# Autodesk Inventor assembly: PreFoldedBody
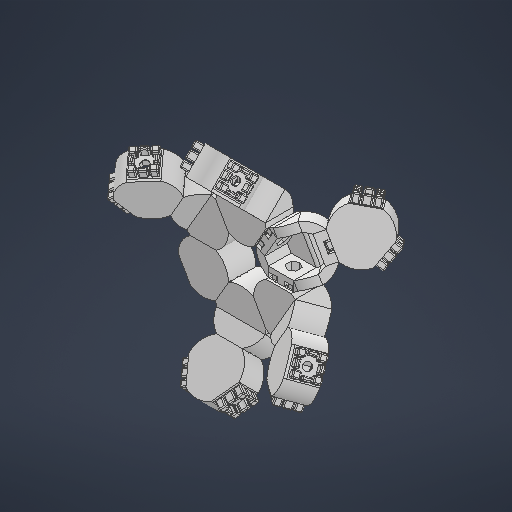
[picture p0: Inventor's stored thumbnail of the model, 512x512]
Saved by Autodesk Inventor 2026.2 (Build 302298000, 298)
## iProperties
Created: 2026-04-30
Part Number: PreFoldedBody
Document SubType Name: Assembly
Designer: Jakub Schmidt
Author: Jakub Schmidt
## Documents named in this file (7)
- C:\Users\Jakub Schmidt\Desktop\100M_SA\SG\10mm (Recent)\2x2mm(Recent)\2DFolded\BeetleDarhani\BeetleFold.iam
- C:\Users\Jakub Schmidt\Desktop\100M_SA\SG\10mm (Recent)\2x2mm(Recent)\2DFolded\BeetleDarhani\BodyFoldedSide1.ipt
- C:\Users\Jakub Schmidt\Desktop\100M_SA\SG\10mm (Recent)\2x2mm(Recent)\2DFolded\BeetleDarhani\BodyFoldedSide2.ipt
- C:\Users\Jakub Schmidt\Desktop\100M_SA\SG\10mm (Recent)\2x2mm(Recent)\2DFolded\BeetleDarhani\SGA.ipt
- C:\Users\Jakub Schmidt\Desktop\100M_SA\SG\10mm (Recent)\2x2mm(Recent)\2DFolded\BeetleDarhani\SGB.ipt
- C:\Users\Jakub Schmidt\Desktop\100M_SA\SG\10mm (Recent)\2x2mm(Recent)\2DFolded\BeetleDarhani\Body.ipt
- C:\Users\Jakub Schmidt\Desktop\100M_SA\SG\10mm (Recent)\2x2mm(Recent)\2DFolded\BeetleDarhani\SGX.ipt
## Components (49 placed, 6 different names)
1. BodyFoldedSide1:1 — Mate:1, Mate:2, Mate:3, Mate:16, Mate:17, Mate:18, Flush:1, Mate:78, Mate:79, Mate:80
2. BodyFoldedSide2:1 — Mate:1, Mate:2, Mate:3, Mate:19, Mate:20, Mate:21, Flush:15
3. BodyFoldedSide1:2 — Mate:62, Mate:63, Mate:64, Mate:65, Mate:66, Mate:67
4. BodyFoldedSide2:2 — Mate:85, Mate:86, Mate:87, Flush:10, Flush:11
5. BodyFoldedSide1:3 — Mate:52, Mate:53, Mate:54, Mate:56, Mate:57, Mate:58, Mate:68
6. BodyFoldedSide2:3 — Mate:59, Mate:60, Mate:61, Flush:12
7. BodyFoldedSide1:4 — Mate:22, Mate:23, Mate:24, Flush:1, Mate:26, Mate:27, Mate:30, Flush:3
8. BodyFoldedSide2:4 — Mate:28, Mate:29, Mate:31, Flush:21
9. BodyFoldedSide1:5 — Mate:69, Mate:70, Mate:71, Mate:73, Mate:74, Mate:75
10. BodyFoldedSide2:5 — Mate:82, Mate:83, Mate:84, Flush:19
11. SGA:1 — Flush:2, Mate:78, Mate:79, Mate:80, Mate:81
12. SGB:1 — Mate:16, Mate:17, Mate:18, Mate:77, Flush:9
13. SGB:2 — Mate:19, Mate:20, Mate:21, Flush:14, Mate:117
14. SGB:3 — Mate:22, Mate:23, Mate:24, Flush:2, Mate:81
15. SGA:2 — Mate:26, Mate:27, Mate:30, Mate:41, Flush:4
16. SGA:3 — Mate:28, Mate:29, Mate:31, Flush:20, Mate:138
17. Body:1 — Mate:32, Mate:33, Mate:34, Mate:35, Mate:36, Mate:37, Mate:38, Mate:39, Mate:40, Flush:3
18. SGB:4 — Mate:33, Mate:34, Mate:39, Mate:72, Flush:5, Flush:6
19. SGB:5 — Mate:32, Mate:35, Mate:40, Mate:41, Flush:4
20. SGA:4 — Mate:36, Mate:37, Mate:38
21. SGA:7 — Mate:52, Mate:53, Mate:54, Flush:7, Flush:8, Mate:76
22. SGB:7 — Mate:56, Mate:57, Mate:58
23. SGB:8 — Mate:59, Mate:60, Mate:61, Mate:116, Flush:13
24. SGA:8 — Mate:65, Mate:66, Mate:67, Mate:68
25. SGA:9 — Mate:62, Mate:63, Mate:64, Mate:77, Flush:9
26. SGA:10 — Mate:69, Mate:70, Mate:71, Mate:72, Flush:5, Flush:6
27. SGB:9 — Mate:73, Mate:74, Mate:75, Flush:7, Flush:8, Mate:76
28. SGA:11 — Mate:82, Mate:83, Mate:84, Flush:18, Mate:137
29. SGB:10 — Mate:85, Mate:86, Mate:87, Mate:97
30. Body:2 — Mate:88, Mate:89, Mate:90, Mate:91, Mate:92, Mate:93, Mate:94, Mate:95, Mate:96, Flush:11
31. SGA:12 — Mate:88, Mate:89, Mate:90, Mate:97, Flush:10
32. SGX:1 — Mate:91, Mate:92, Mate:93
33. SGX:2 — Mate:94, Mate:95, Mate:96
34. Body:3 — Flush:12
35. SGA:13 — Mate:116, Flush:13
36. SGX:3
37. SGX:4
38. Body:4 — Flush:15
39. SGA:14 — Flush:14, Mate:117
40. SGX:5
41. SGX:6
42. Body:5 — Mate:127, Mate:128, Flush:16, Flush:19
43. SGX:7
44. SGX:8
45. SGB:11 — Mate:127, Mate:128, Flush:16, Flush:18, Mate:137
46. Body:6 — Flush:21
47. SGX:9
48. SGX:10
49. SGB:12 — Flush:20, Mate:138
## Relationships (144: Mate 123, Flush 21)
- Mate:1: BodyFoldedSide1:1 ↔ BodyFoldedSide2:1
- Mate:2: BodyFoldedSide1:1 ↔ BodyFoldedSide2:1
- Mate:3: BodyFoldedSide1:1 ↔ BodyFoldedSide2:1
- [Mate]: BodyFoldedSide1:2 ↔ BodyFoldedSide2:2
- [Mate]: BodyFoldedSide1:2 ↔ BodyFoldedSide2:2
- [Mate]: BodyFoldedSide1:2 ↔ BodyFoldedSide2:2
- [Mate]: BodyFoldedSide1:3 ↔ BodyFoldedSide2:3
- [Mate]: BodyFoldedSide1:3 ↔ BodyFoldedSide2:3
- [Mate]: BodyFoldedSide1:3 ↔ BodyFoldedSide2:3
- [Mate]: BodyFoldedSide1:4 ↔ BodyFoldedSide2:4
- [Mate]: BodyFoldedSide1:4 ↔ BodyFoldedSide2:4
- [Mate]: BodyFoldedSide1:4 ↔ BodyFoldedSide2:4
- [Mate]: BodyFoldedSide1:5 ↔ BodyFoldedSide2:5
- [Mate]: BodyFoldedSide1:5 ↔ BodyFoldedSide2:5
- [Mate]: BodyFoldedSide1:5 ↔ BodyFoldedSide2:5
- Mate:16: BodyFoldedSide1:1 ↔ SGB:1
- Mate:17: BodyFoldedSide1:1 ↔ SGB:1
- Mate:18: BodyFoldedSide1:1 ↔ SGB:1
- Mate:19: BodyFoldedSide2:1 ↔ SGB:2
- Mate:20: BodyFoldedSide2:1 ↔ SGB:2
- Mate:21: BodyFoldedSide2:1 ↔ SGB:2
- Mate:22: BodyFoldedSide1:4 ↔ SGB:3
- Mate:23: BodyFoldedSide1:4 ↔ SGB:3
- Mate:24: BodyFoldedSide1:4 ↔ SGB:3
- Flush:1: BodyFoldedSide1:1 ↔ BodyFoldedSide1:4
- Flush:2: SGA:1 ↔ SGB:3
- Mate:26: BodyFoldedSide1:4 ↔ SGA:2
- Mate:27: BodyFoldedSide1:4 ↔ SGA:2
- Mate:28: BodyFoldedSide2:4 ↔ SGA:3
- Mate:29: BodyFoldedSide2:4 ↔ SGA:3
- Mate:30: BodyFoldedSide1:4 ↔ SGA:2
- Mate:31: BodyFoldedSide2:4 ↔ SGA:3
- Mate:32: Body:1 ↔ SGB:5
- Mate:33: Body:1 ↔ SGB:4
- Mate:34: Body:1 ↔ SGB:4
- Mate:35: Body:1 ↔ SGB:5
- Mate:36: Body:1 ↔ SGA:4
- Mate:37: Body:1 ↔ SGA:4
- Mate:38: Body:1 ↔ SGA:4
- Mate:39: Body:1 ↔ SGB:4
- Mate:40: Body:1 ↔ SGB:5
- Mate:41: SGA:2 ↔ SGB:5
- Flush:3: BodyFoldedSide1:4 ↔ Body:1
- Flush:4: SGA:2 ↔ SGB:5
- Mate:52: BodyFoldedSide1:3 ↔ SGA:7
- Mate:53: BodyFoldedSide1:3 ↔ SGA:7
- Mate:54: BodyFoldedSide1:3 ↔ SGA:7
- Mate:56: BodyFoldedSide1:3 ↔ SGB:7
- Mate:57: BodyFoldedSide1:3 ↔ SGB:7
- Mate:58: BodyFoldedSide1:3 ↔ SGB:7
- Mate:59: BodyFoldedSide2:3 ↔ SGB:8
- Mate:60: BodyFoldedSide2:3 ↔ SGB:8
- Mate:61: BodyFoldedSide2:3 ↔ SGB:8
- Mate:62: BodyFoldedSide1:2 ↔ SGA:9
- Mate:63: BodyFoldedSide1:2 ↔ SGA:9
- Mate:64: BodyFoldedSide1:2 ↔ SGA:9
- Mate:65: BodyFoldedSide1:2 ↔ SGA:8
- Mate:66: BodyFoldedSide1:2 ↔ SGA:8
- Mate:67: BodyFoldedSide1:2 ↔ SGA:8
- Mate:68: BodyFoldedSide1:3 ↔ SGA:8
- Mate:69: BodyFoldedSide1:5 ↔ SGA:10
- Mate:70: BodyFoldedSide1:5 ↔ SGA:10
- Mate:71: BodyFoldedSide1:5 ↔ SGA:10
- Mate:72: SGB:4 ↔ SGA:10
- Flush:5: SGB:4 ↔ SGA:10
- Flush:6: SGB:4 ↔ SGA:10
- Mate:73: BodyFoldedSide1:5 ↔ SGB:9
- Mate:74: BodyFoldedSide1:5 ↔ SGB:9
- Mate:75: BodyFoldedSide1:5 ↔ SGB:9
- Flush:7: SGA:7 ↔ SGB:9
- Flush:8: SGA:7 ↔ SGB:9
- Mate:76: SGA:7 ↔ SGB:9
- Mate:77: SGB:1 ↔ SGA:9
- Mate:78: BodyFoldedSide1:1 ↔ SGA:1
- Mate:79: BodyFoldedSide1:1 ↔ SGA:1
- Mate:80: BodyFoldedSide1:1 ↔ SGA:1
- Mate:81: SGA:1 ↔ SGB:3
- Flush:9: SGB:1 ↔ SGA:9
- Mate:82: BodyFoldedSide2:5 ↔ SGA:11
- Mate:83: BodyFoldedSide2:5 ↔ SGA:11
- Mate:84: BodyFoldedSide2:5 ↔ SGA:11
- Mate:85: BodyFoldedSide2:2 ↔ SGB:10
- Mate:86: BodyFoldedSide2:2 ↔ SGB:10
- Mate:87: BodyFoldedSide2:2 ↔ SGB:10
- Mate:88: Body:2 ↔ SGA:12
- Mate:89: Body:2 ↔ SGA:12
- Mate:90: Body:2 ↔ SGA:12
- Mate:91: Body:2 ↔ SGX:1
- Mate:92: Body:2 ↔ SGX:1
- Mate:93: Body:2 ↔ SGX:1
- Mate:94: Body:2 ↔ SGX:2
- Mate:95: Body:2 ↔ SGX:2
- Mate:96: Body:2 ↔ SGX:2
- Mate:97: SGB:10 ↔ SGA:12
- Flush:10: BodyFoldedSide2:2 ↔ SGA:12
- Flush:11: BodyFoldedSide2:2 ↔ Body:2
- [Mate]: Body:3 ↔ SGA:13
- [Mate]: Body:3 ↔ SGA:13
- [Mate]: Body:3 ↔ SGA:13
- [Mate]: Body:3 ↔ SGX:3
- [Mate]: Body:3 ↔ SGX:3
- [Mate]: Body:3 ↔ SGX:3
- [Mate]: Body:3 ↔ SGX:4
- [Mate]: Body:3 ↔ SGX:4
- [Mate]: Body:3 ↔ SGX:4
- [Mate]: Body:4 ↔ SGA:14
- [Mate]: Body:4 ↔ SGA:14
- [Mate]: Body:4 ↔ SGA:14
- [Mate]: Body:4 ↔ SGX:5
- [Mate]: Body:4 ↔ SGX:5
- [Mate]: Body:4 ↔ SGX:5
- [Mate]: Body:4 ↔ SGX:6
- [Mate]: Body:4 ↔ SGX:6
- [Mate]: Body:4 ↔ SGX:6
- Mate:116: SGB:8 ↔ SGA:13
- Flush:12: BodyFoldedSide2:3 ↔ Body:3
- Flush:13: SGB:8 ↔ SGA:13
- Flush:14: SGB:2 ↔ SGA:14
- Mate:117: SGB:2 ↔ SGA:14
- Flush:15: BodyFoldedSide2:1 ↔ Body:4
- [Mate]: Body:5 ↔ SGX:7
- [Mate]: Body:5 ↔ SGX:7
- [Mate]: Body:5 ↔ SGX:7
- [Mate]: Body:5 ↔ SGX:8
- [Mate]: Body:5 ↔ SGX:8
- [Mate]: Body:5 ↔ SGX:8
- Mate:127: Body:5 ↔ SGB:11
- Mate:128: Body:5 ↔ SGB:11
- Flush:16: Body:5 ↔ SGB:11
- [Mate]: Body:6 ↔ SGX:9
- [Mate]: Body:6 ↔ SGX:9
- [Mate]: Body:6 ↔ SGX:9
- [Mate]: Body:6 ↔ SGX:10
- [Mate]: Body:6 ↔ SGX:10
- [Mate]: Body:6 ↔ SGX:10
- [Mate]: Body:6 ↔ SGB:12
- [Mate]: Body:6 ↔ SGB:12
- [Flush]: Body:6 ↔ SGB:12
- Flush:18: SGA:11 ↔ SGB:11
- Mate:137: SGA:11 ↔ SGB:11
- Flush:19: BodyFoldedSide2:5 ↔ Body:5
- Flush:20: SGA:3 ↔ SGB:12
- Mate:138: SGA:3 ↔ SGB:12
- Flush:21: BodyFoldedSide2:4 ↔ Body:6
## Named parameters: d3_d0 = 0 mm, d4_d1 = 0 mm, d5_d2 = 0 mm, d6_d0 = 0 mm, d7_d1 = 0 mm, d8_d2 = 0 mm, d9_d0 = 0 mm, d10_d1 = 0 mm, d11_d2 = 0 mm, d12_d0 = 0 mm, d13_d1 = 0 mm, d14_d2 = 0 mm, d113_d101 = 0 mm, d114_d102 = 0 mm, d115_d103 = 0 mm, d116_d104 = 0 mm, d117_d105 = 0 mm, d118_d106 = 0 mm, d119_d107 = 0 mm, d120_d108 = 0 mm, d121_d109 = 0 mm, d122_d101 = 0 mm, d123_d102 = 0 mm, d124_d103 = 0 mm, d125_d104 = 0 mm, d126_d105 = 0 mm, d127_d106 = 0 mm, d128_d107 = 0 mm, d129_d108 = 0 mm, d130_d109 = 0 mm, d140_d104 = 0 mm, d141_d105 = 0 mm, d142_d106 = 0 mm, d143_d107 = 0 mm, d144_d108 = 0 mm, d145_d109 = 0 mm, d149_d140_d104 = 0 mm, d150_d141_d105 = 0 mm, d151_d142_d106 = 0 mm, d152_d143_d107 = 0 mm, d153_d144_d108 = 0 mm, d154_d145_d109 = 0 mm, d155_d146 = 0 mm, d156_d147 = 0 mm, d157_d148 = 0 mm
